# Autodesk Inventor assembly: Right Side
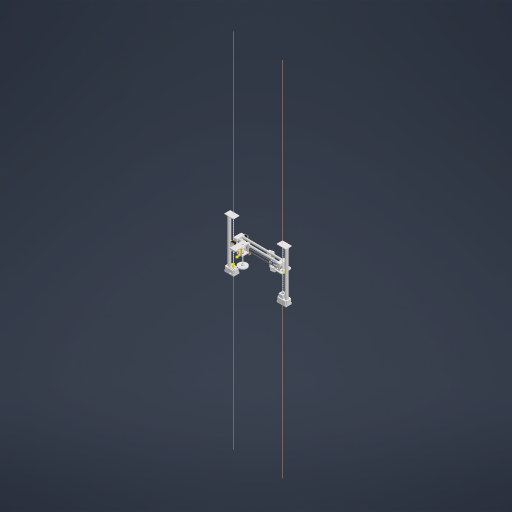
[picture p0: Inventor's stored thumbnail of the model, 512x512]
Saved by Autodesk Inventor 2024.2 (Build 282272000, 272)
## iProperties
Created: 2024-03-21
Part Number: Right Side
Document SubType Name: Assembly
Designer: LightStore
Author: LightStore
## Documents named in this file (25)
- C:\Users\seifs\Downloads\Final Assembly\Main Assembly.iam
- C:\Users\seifs\Downloads\Final Assembly\LeadNut.ipt
- C:\Users\seifs\Downloads\Final Assembly\LeadScrew1.ipt
- C:\Users\seifs\Downloads\Final Assembly\midle part right.ipt
- C:\Users\seifs\Downloads\Final Assembly\project_base_right.ipt
- C:\Users\seifs\Downloads\Final Assembly\pvc.ipt
- C:\Users\seifs\Downloads\Final Assembly\Rolling bearing B708 C GB_T 292-2007.ipt
- C:\Users\seifs\Downloads\Final Assembly\Top_part.ipt
- C:\Users\seifs\Downloads\Final Assembly\ISO 4036 - M3(2).ipt
- C:\Users\seifs\Downloads\Final Assembly\ISO 7046-1 - M3 x 20_ - 4.8 - Z - ISO.ipt
- C:\Users\seifs\Downloads\Final Assembly\V-Belt transmission4.iam
- C:\Users\seifs\Downloads\Final Assembly\Beltclamp.ipt
- C:\Users\seifs\Downloads\Final Assembly\pvc middle.ipt
- C:\Users\seifs\Downloads\Final Assembly\Assembly_motorcoverbase.iam
- C:\Users\seifs\Downloads\Final Assembly\Assembly_motorcoverbase_2.iam
- C:\Users\seifs\Downloads\Final Assembly\brush end effector.iam
- C:\Users\seifs\Downloads\Final Assembly\brush end effector_2.iam
- C:\Users\seifs\Downloads\Final Assembly\brush end effector_3.iam
- C:\Users\seifs\Downloads\Final Assembly\FlyCutterSub (1).iam
- C:\Users\seifs\Downloads\Final Assembly\ISO 7046-1 - M3 x 30_ - 4.8 - Z - ISO.ipt
- C:\Users\seifs\Downloads\Final Assembly\ISO 7046-1 - M1.6 x 10_ - 4.8 - Z - ISO.ipt
- C:\Users\seifs\OneDrive\Documents\Inventor\Content Center Files\R2024\en-US\ISO 7046-1 Z(1)\ISO 7046-1 - M3 x 12_ - 4.8 - Z - ISO.ipt
- C:\Users\seifs\OneDrive\Documents\Inventor\Content Center Files\R2024\en-US\ISO 7046-1 Z(1)\ISO 7046-1 - M3 x 20_ - 4.8 - Z - ISO.ipt
- C:\Users\seifs\Downloads\Final Assembly\V-Belt transmission4_MIR.iam
- C:\Users\seifs\Downloads\Final Assembly\pvc middle_MIR.ipt
## Components (45 placed, 23 different names)
1. midle part right:1 — Rotational:1, Rotational:2, Insert:9, Insert:10, Insert:11, Insert:12, Insert:16, Insert:18, Angle:1, Mate:15, Insert:44, Insert:45
2. project_base_right:1 — Insert:1, Insert:3, Angle:1, Angle:2, Angle:3
3. pvc:1 — Insert:1, Mate:2
4. Bearing GB/T 292-2007 Type IN - withdrawn B708 C:1 — Insert:5, Insert:6
5. Bearing GB/T 292-2007 Type IN - withdrawn B708 C:2 — Insert:3, Insert:4
6. LeadScrew1:1 — Insert:4, Insert:5, Mate:1
7. Top_part:1 — Insert:6, Mate:2
8. LeadNut:1 — Rotational:1, Rotational:2, Mate:1, Insert:8, Insert:13, Insert:14, Insert:15
9. ISO 4036 M3:1 — Insert:8
10. ISO 7046-1 Z M3 x 20 - 4.8 - Z:1 — Insert:12
11. ISO 7046-1 Z M3 x 20 - 4.8 - Z:2 — Insert:10
12. ISO 7046-1 Z M3 x 20 - 4.8 - Z:3 — Insert:11
13. ISO 7046-1 Z M3 x 20 - 4.8 - Z:4 — Insert:9
14. ISO 4036 M3:2 — Insert:13
15. ISO 4036 M3:3 — Insert:14
16. ISO 4036 M3:4 — Insert:15
17. Bearing GB/T 292-2007 Type IN - withdrawn B708 C:3 — Insert:16, Insert:17
18. V-Belt transmission:1 [sub-assembly] — Insert:17, Mate:7, Mate:18, Mate:19
19. pvc middle:1 — Insert:18
20. Assembly_motorcoverbase:1 [sub-assembly] — Mate:7, Mate:9, Mate:16
21. Assembly_motorcoverbase_2:1 [sub-assembly] — Mate:9, Angle:2, Angle:3
22. brush end effector:1 [sub-assembly] — Insert:21, Insert:26, Insert:27, Insert:28, Insert:29, Insert:46, Insert:47
23. brush end effector_2:1 [sub-assembly] — Insert:21, Insert:22, Insert:23
24. brush end effector_3:1 [sub-assembly] — Insert:22, Insert:23
25. ISO 7046-1 Z M3 x 30 - 4.8 - Z:1 — Insert:27
26. ISO 7046-1 Z M3 x 30 - 4.8 - Z:2 — Insert:28
27. ISO 7046-1 Z M3 x 30 - 4.8 - Z:3 — Insert:26
28. ISO 7046-1 Z M3 x 30 - 4.8 - Z:4 — Insert:29
29. ISO 7046-1 Z M1.6 x 10 - 4.8 - Z:1 — Insert:37
30. ISO 7046-1 Z M1.6 x 10 - 4.8 - Z:2 — Insert:39
31. ISO 7046-1 Z M1.6 x 10 - 4.8 - Z:3 — Insert:36
32. ISO 7046-1 Z M1.6 x 10 - 4.8 - Z:4 — Insert:38
33. FlyCutterSub (1):1 [sub-assembly] — Insert:32, Insert:33, Insert:34, Insert:35, Insert:36, Insert:37, Insert:38, Insert:39, Insert:40, Insert:41, Insert:42, Insert:48, Insert:49
34. ISO 7046-1 Z M3 x 30 - 4.8 - Z:5 — Insert:34
35. ISO 7046-1 Z M3 x 30 - 4.8 - Z:6 — Insert:35
36. ISO 7046-1 Z M3 x 30 - 4.8 - Z:7 — Insert:33
37. ISO 7046-1 Z M3 x 30 - 4.8 - Z:8 — Insert:32
38. ISO 7046-1 Z M3 x 20 - 4.8 - Z:5 — Insert:40
39. ISO 7046-1 Z M3 x 12 - 4.8 - Z:1 — Insert:41
40. ISO 7046-1 Z M3 x 12 - 4.8 - Z:2 — Insert:42
41. Bearing GB/T 292-2007 Type IN - withdrawn B708 C:4 — Insert:43, Mate:15
42. V-Belt transmission4_MIR:1 [sub-assembly] — Insert:43, Insert:44, Mate:16, Mate:17, Mate:20, Mate:21
43. pvc middle_MIR:1 — Insert:45
44. Beltclamp:1 — Mate:17, Mate:18, Mate:19, Insert:48, Insert:49
45. Beltclamp:2 — Mate:20, Mate:21, Insert:46, Insert:47
## Relationships (57: Insert 41, Mate 11, Angle 3, RevoluteJoint 2)
- Insert:1: project_base_right:1 ↔ pvc:1
- Insert:3: project_base_right:1 ↔ Bearing GB/T 292-2007 Type IN - withdrawn B708 C:2
- Insert:4: Bearing GB/T 292-2007 Type IN - withdrawn B708 C:2 ↔ LeadScrew1:1
- Insert:5: Bearing GB/T 292-2007 Type IN - withdrawn B708 C:1 ↔ LeadScrew1:1
- Insert:6: Bearing GB/T 292-2007 Type IN - withdrawn B708 C:1 ↔ Top_part:1
- Rotational:1 [RevoluteJoint]: midle part right:1 ↔ LeadNut:1
- Rotational:2 [RevoluteJoint]: midle part right:1 ↔ LeadNut:1
- Mate:1: LeadScrew1:1 ↔ LeadNut:1
- Mate:2: pvc:1 ↔ Top_part:1
- Insert:8: LeadNut:1 ↔ ISO 4036 M3:1
- Insert:9: midle part right:1 ↔ ISO 7046-1 Z M3 x 20 - 4.8 - Z:4
- Insert:10: midle part right:1 ↔ ISO 7046-1 Z M3 x 20 - 4.8 - Z:2
- Insert:11: midle part right:1 ↔ ISO 7046-1 Z M3 x 20 - 4.8 - Z:3
- Insert:12: midle part right:1 ↔ ISO 7046-1 Z M3 x 20 - 4.8 - Z:1
- Insert:13: LeadNut:1 ↔ ISO 4036 M3:2
- Insert:14: LeadNut:1 ↔ ISO 4036 M3:3
- Insert:15: LeadNut:1 ↔ ISO 4036 M3:4
- Insert:16: midle part right:1 ↔ Bearing GB/T 292-2007 Type IN - withdrawn B708 C:3
- Insert:17: Bearing GB/T 292-2007 Type IN - withdrawn B708 C:3 ↔ V-Belt transmission:1
- Insert:18: midle part right:1 ↔ pvc middle:1
- Mate:7: V-Belt transmission:1 ↔ Assembly_motorcoverbase:1
- Mate:9: Assembly_motorcoverbase:1 ↔ Assembly_motorcoverbase_2:1
- Insert:21: brush end effector:1 ↔ brush end effector_2:1
- Insert:22: brush end effector_2:1 ↔ brush end effector_3:1
- Insert:23: brush end effector_2:1 ↔ brush end effector_3:1
- Insert:26: brush end effector:1 ↔ ISO 7046-1 Z M3 x 30 - 4.8 - Z:3
- Insert:27: brush end effector:1 ↔ ISO 7046-1 Z M3 x 30 - 4.8 - Z:1
- Insert:28: brush end effector:1 ↔ ISO 7046-1 Z M3 x 30 - 4.8 - Z:2
- Insert:29: brush end effector:1 ↔ ISO 7046-1 Z M3 x 30 - 4.8 - Z:4
- Angle:1 (0 deg): midle part right:1 ↔ project_base_right:1
- Angle:2 (0 deg): project_base_right:1 ↔ Assembly_motorcoverbase_2:1
- Angle:3 (0 deg): project_base_right:1 ↔ Assembly_motorcoverbase_2:1
- Insert:32: FlyCutterSub (1):1 ↔ ISO 7046-1 Z M3 x 30 - 4.8 - Z:8
- Insert:33: FlyCutterSub (1):1 ↔ ISO 7046-1 Z M3 x 30 - 4.8 - Z:7
- Insert:34: FlyCutterSub (1):1 ↔ ISO 7046-1 Z M3 x 30 - 4.8 - Z:5
- Insert:35: FlyCutterSub (1):1 ↔ ISO 7046-1 Z M3 x 30 - 4.8 - Z:6
- Insert:36: ISO 7046-1 Z M1.6 x 10 - 4.8 - Z:3 ↔ FlyCutterSub (1):1
- Insert:37: ISO 7046-1 Z M1.6 x 10 - 4.8 - Z:1 ↔ FlyCutterSub (1):1
- Insert:38: ISO 7046-1 Z M1.6 x 10 - 4.8 - Z:4 ↔ FlyCutterSub (1):1
- Insert:39: ISO 7046-1 Z M1.6 x 10 - 4.8 - Z:2 ↔ FlyCutterSub (1):1
- Insert:40: FlyCutterSub (1):1 ↔ ISO 7046-1 Z M3 x 20 - 4.8 - Z:5
- Insert:41: FlyCutterSub (1):1 ↔ ISO 7046-1 Z M3 x 12 - 4.8 - Z:1
- Insert:42: FlyCutterSub (1):1 ↔ ISO 7046-1 Z M3 x 12 - 4.8 - Z:2
- Insert:43: Bearing GB/T 292-2007 Type IN - withdrawn B708 C:4 ↔ V-Belt transmission4_MIR:1
- Mate:15: midle part right:1 ↔ Bearing GB/T 292-2007 Type IN - withdrawn B708 C:4
- Insert:44: midle part right:1 ↔ V-Belt transmission4_MIR:1
- Mate:16: Assembly_motorcoverbase:1 ↔ V-Belt transmission4_MIR:1
- Insert:45: midle part right:1 ↔ pvc middle_MIR:1
- Mate:17: V-Belt transmission4_MIR:1 ↔ Beltclamp:1
- Mate:18: V-Belt transmission:1 ↔ Beltclamp:1
- Mate:19: V-Belt transmission:1 ↔ Beltclamp:1
- Mate:20: V-Belt transmission4_MIR:1 ↔ Beltclamp:2
- Mate:21: V-Belt transmission4_MIR:1 ↔ Beltclamp:2
- Insert:46: brush end effector:1 ↔ Beltclamp:2
- Insert:47: brush end effector:1 ↔ Beltclamp:2
- Insert:48: FlyCutterSub (1):1 ↔ Beltclamp:1
- Insert:49: FlyCutterSub (1):1 ↔ Beltclamp:1
